# Autodesk Inventor assembly: aseembly
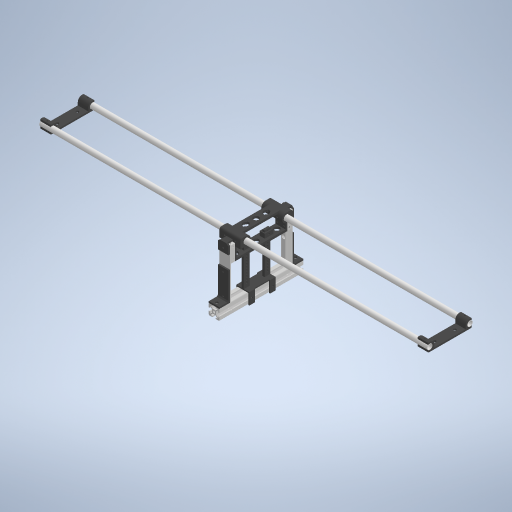
[picture p0: Inventor's stored thumbnail of the model, 512x512]
Saved by Autodesk Inventor 2024 (Build 280153000, 153)
## iProperties
Created: 2024-09-08
Part Number: aseembly
Document SubType Name: Assembly
Designer: Gihyeok
Author: Gihyeok
## Documents named in this file (9)
- D:\OneDrive\Tokyo Tech\Project\Dog Robot\Hoshiramu_robot\component\linear_guide\aseembly.iam
- D:\OneDrive\Tokyo Tech\Project\Dog Robot\Hoshiramu_robot\component\linear_guide\HFS5-2020-160-AH24-BH136-Z6-XA20-XB65-XC140_Autodesk_Inventor_2024_20240908\HFS5-2020-160-AH24-BH136-Z6-XA20-XB65-XC140.ipt
- D:\OneDrive\Tokyo Tech\Project\Dog Robot\Hoshiramu_robot\component\linear_guide\base.ipt
- D:\OneDrive\Tokyo Tech\Project\Dog Robot\Hoshiramu_robot\component\linear_guide\linear_rail(JKSG10-95-S1)\JKSG10-95-S1.iam
- D:\OneDrive\Tokyo Tech\Project\Dog Robot\Hoshiramu_robot\component\linear_guide\top.ipt
- D:\OneDrive\Tokyo Tech\Project\Dog Robot\Hoshiramu_robot\component\linear_guide\catcher_2ea.ipt
- D:\OneDrive\Tokyo Tech\Project\Dog Robot\Hoshiramu_robot\component\linear_guide\latch.ipt
- D:\OneDrive\Tokyo Tech\Project\Dog Robot\Hoshiramu_robot\component\linear_guide\aluminium_pipe_10mm_740mm.ipt
- D:\OneDrive\Tokyo Tech\Project\Dog Robot\Hoshiramu_robot\component\linear_guide\pipe_holder.ipt
## Components (13 placed, 8 different names)
1. HFS5-2020-160-AH24-BH136-Z6-XA20-XB65-XC140:1 — 메이트:17, 메이트:18, 플러쉬:2, 메이트:19, 메이트:20
2. base:1 — 메이트:14, 메이트:15, 메이트:16
3. base:2 — 메이트:11, 메이트:12, 메이트:13, 메이트:17, 메이트:18, 플러쉬:2
4. JKSG10-95-S1:2 [sub-assembly] — 메이트:1, 메이트:2, 메이트:6, 메이트:9, 메이트:10, 플러쉬:1, 메이트:14, 메이트:15, 메이트:16
5. top:1 — 메이트:1, 메이트:2, 메이트:3, 메이트:4, 메이트:5, 메이트:6, 메이트:21, 메이트:22, 메이트:23, 메이트:24, 메이트:25
6. JKSG10-95-S1:3 [sub-assembly] — 메이트:3, 메이트:4, 메이트:5, 메이트:7, 메이트:8, 메이트:11, 메이트:12, 메이트:13
7. catcher_2ea:1 — 메이트:19, 메이트:20, 메이트:21
8. latch:1 — 메이트:7, 메이트:8
9. latch:2 — 메이트:9, 메이트:10, 플러쉬:1
10. aluminium_pipe_10mm_740mm:1 — 메이트:22, 메이트:23, 메이트:28, 메이트:29
11. aluminium_pipe_10mm_740mm:2 — 메이트:24, 메이트:25, 메이트:26, 메이트:27
12. pipe_holder:1 — 메이트:26, 메이트:27
13. pipe_holder:2 — 메이트:28, 메이트:29
## Relationships (31: Mate 29, Flush 2)
- 메이트:1 [Mate]: JKSG10-95-S1:2 ↔ top:1
- 메이트:2 [Mate]: JKSG10-95-S1:2 ↔ top:1
- 메이트:3 [Mate]: top:1 ↔ JKSG10-95-S1:3
- 메이트:4 [Mate]: top:1 ↔ JKSG10-95-S1:3
- 메이트:5 [Mate]: top:1 ↔ JKSG10-95-S1:3
- 메이트:6 [Mate]: JKSG10-95-S1:2 ↔ top:1
- 메이트:7 [Mate]: JKSG10-95-S1:3 ↔ latch:1
- 메이트:8 [Mate]: JKSG10-95-S1:3 ↔ latch:1
- 메이트:9 [Mate]: JKSG10-95-S1:2 ↔ latch:2
- 메이트:10 [Mate]: JKSG10-95-S1:2 ↔ latch:2
- 플러쉬:1 [Flush]: JKSG10-95-S1:2 ↔ latch:2
- 메이트:11 [Mate]: base:2 ↔ JKSG10-95-S1:3
- 메이트:12 [Mate]: base:2 ↔ JKSG10-95-S1:3
- 메이트:13 [Mate]: base:2 ↔ JKSG10-95-S1:3
- 메이트:14 [Mate]: base:1 ↔ JKSG10-95-S1:2
- 메이트:15 [Mate]: base:1 ↔ JKSG10-95-S1:2
- 메이트:16 [Mate]: base:1 ↔ JKSG10-95-S1:2
- 메이트:17 [Mate]: HFS5-2020-160-AH24-BH136-Z6-XA20-XB65-XC140:1 ↔ base:2
- 메이트:18 [Mate]: HFS5-2020-160-AH24-BH136-Z6-XA20-XB65-XC140:1 ↔ base:2
- 플러쉬:2 [Flush]: HFS5-2020-160-AH24-BH136-Z6-XA20-XB65-XC140:1 ↔ base:2
- 메이트:19 [Mate]: HFS5-2020-160-AH24-BH136-Z6-XA20-XB65-XC140:1 ↔ catcher_2ea:1
- 메이트:20 [Mate]: HFS5-2020-160-AH24-BH136-Z6-XA20-XB65-XC140:1 ↔ catcher_2ea:1
- 메이트:21 [Mate]: top:1 ↔ catcher_2ea:1
- 메이트:22 [Mate]: top:1 ↔ aluminium_pipe_10mm_740mm:1
- 메이트:23 [Mate]: top:1 ↔ aluminium_pipe_10mm_740mm:1
- 메이트:24 [Mate]: top:1 ↔ aluminium_pipe_10mm_740mm:2
- 메이트:25 [Mate]: top:1 ↔ aluminium_pipe_10mm_740mm:2
- 메이트:26 [Mate]: aluminium_pipe_10mm_740mm:2 ↔ pipe_holder:1
- 메이트:27 [Mate]: aluminium_pipe_10mm_740mm:2 ↔ pipe_holder:1
- 메이트:28 [Mate]: aluminium_pipe_10mm_740mm:1 ↔ pipe_holder:2
- 메이트:29 [Mate]: aluminium_pipe_10mm_740mm:1 ↔ pipe_holder:2
